# Autodesk Inventor assembly: kezfej_1
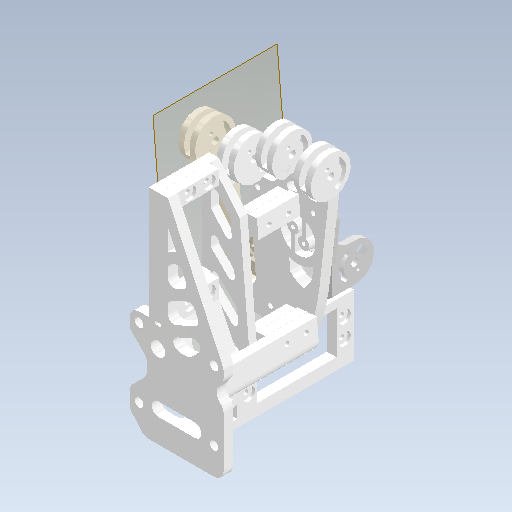
[picture p0: Inventor's stored thumbnail of the model, 512x512]
Saved by Autodesk Inventor 2020.3 (Build 243373000, 373)
## iProperties
Created: 2019-09-26
Part Number: kezfej_1
Document SubType Name: Assembly
Designer: Horváth Patrik
Author: Horváth Patrik
## Documents named in this file (7)
- E:\Dokumentumok\Simonyi\INDACT\Robotarm - kézfej fileok\kéz12.0\kezfej_1.iam
- E:\Dokumentumok\Simonyi\INDACT\Robotarm - kézfej fileok\kéz12.0\Solid1_1.ipt
- E:\Dokumentumok\Simonyi\INDACT\Robotarm - kézfej fileok\kéz12.0\Solid3_1.ipt
- E:\Dokumentumok\Simonyi\INDACT\Robotarm - kézfej fileok\kéz12.0\Solid2_1.ipt
- E:\Dokumentumok\Simonyi\INDACT\Robotarm - kézfej fileok\kéz12.0\Solid4_1.ipt
- E:\Dokumentumok\Simonyi\INDACT\Robotarm - kézfej fileok\kéz12.0\Solid4_11.ipt
- E:\Dokumentumok\Simonyi\INDACT\Robotarm - kézfej fileok\kéz12.0\Solid1_11.ipt
## Components (8 placed, 6 different names)
1. Solid1_1:1 — Mate:1, Mate:2, Mate:3, Symmetry:1, Mate:4, Mate:5, Mate:6, Mate:7, Mate:8, Mate:9, Mate:10, Mate:11, Mate:12, Flush:1
2. Solid3_1:1 — Mate:7, Mate:8, Mate:9
3. Solid2_1:1 — Mate:13, Mate:14, Mate:15, Flush:1
4. Solid4_1:1 — Symmetry:1
5. Solid4_1:2 — Mate:1, Mate:2, Mate:3
6. Solid4_11:1
7. Solid4_11:2 — Mate:4, Mate:5, Mate:6
8. Solid1_11:1 — Mate:10, Mate:11, Mate:12, Mate:13, Mate:14, Mate:15
## Relationships (17: Mate 15, Symmetry 1, Flush 1)
- Mate:1: Solid1_1:1 ↔ Solid4_1:2
- Mate:2: Solid1_1:1 ↔ Solid4_1:2
- Mate:3: Solid1_1:1 ↔ Solid4_1:2
- Symmetry:1: Solid1_1:1 ↔ Solid4_1:1
- Mate:4: Solid1_1:1 ↔ Solid4_11:2
- Mate:5: Solid1_1:1 ↔ Solid4_11:2
- Mate:6: Solid1_1:1 ↔ Solid4_11:2
- Mate:7: Solid1_1:1 ↔ Solid3_1:1
- Mate:8: Solid1_1:1 ↔ Solid3_1:1
- Mate:9: Solid1_1:1 ↔ Solid3_1:1
- Mate:10: Solid1_1:1 ↔ Solid1_11:1
- Mate:11: Solid1_1:1 ↔ Solid1_11:1
- Mate:12: Solid1_1:1 ↔ Solid1_11:1
- Mate:13: Solid2_1:1 ↔ Solid1_11:1
- Mate:14: Solid2_1:1 ↔ Solid1_11:1
- Mate:15: Solid2_1:1 ↔ Solid1_11:1
- Flush:1: Solid1_1:1 ↔ Solid2_1:1
